# Autodesk Inventor assembly: 4461-17-0101 + Bearing
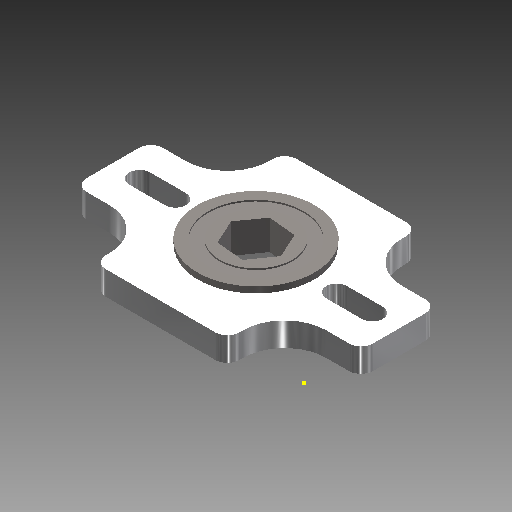
[picture p0: Inventor's stored thumbnail of the model, 512x512]
Saved by Autodesk Inventor 2018 (Build 220112000, 112)
## iProperties
Created: 2017-12-14
Part Number: 4461-17-0101 + Bearing
Document SubType Name: Assembly
Designer: S-2512711
Author: S-2512711
## Documents named in this file (3)
- C:\Users\S-2512711\Desktop\Drivebase 2018 Files Final Kinda\Drivebase 2018 Files Final Kinda\Drivebase 2018 Files 2\Drivebase 2018 Files 2\4461-17-0101 + Bearing.iam
- C:\Users\S-2512711\Desktop\Drivebase 2018 Files Final Kinda\Drivebase 2018 Files Final Kinda\Drivebase 2018 Files 2\Drivebase 2018 Files 2\4461-17-0101 Tensioner Plate.ipt
- C:\Users\S-2512711\Desktop\Drivebase 2018 Files Final Kinda\Drivebase 2018 Files Final Kinda\Drivebase 2018 Files 2\Drivebase 2018 Files 2\0_500_Hex_ID_x_1_125_OD_x_0_313_WD_Flanged_Bearing_v2_217-3875.ipt
## Components (2 placed, 2 different names)
1. 4461-17-0101 Tensioner Plate:1 — Mate:1, Mate:2, Rotation:1
2. 0_500_Hex_ID_x_1_125_OD_x_0_313_WD_Flanged_Bearing_v2_217-3875:1 — Mate:1, Mate:2, Rotation:1
## Relationships (3: Mate 2, RelateRotation 1)
- Mate:1: 4461-17-0101 Tensioner Plate:1 ↔ 0_500_Hex_ID_x_1_125_OD_x_0_313_WD_Flanged_Bearing_v2_217-3875:1
- Mate:2: 4461-17-0101 Tensioner Plate:1 ↔ 0_500_Hex_ID_x_1_125_OD_x_0_313_WD_Flanged_Bearing_v2_217-3875:1
- Rotation:1 [RelateRotation] (1 ul): 4461-17-0101 Tensioner Plate:1 ↔ 0_500_Hex_ID_x_1_125_OD_x_0_313_WD_Flanged_Bearing_v2_217-3875:1
